# Autodesk Inventor assembly: A2017_T2_05
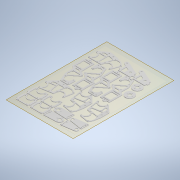
[picture p0: Inventor's stored thumbnail of the model, 180x180]
Saved by Autodesk Inventor 2020 (Build 240168000, 168)
## iProperties
Created: 2021-08-27
Part Number: A2017_T2_05
Document SubType Name: Assembly
Designer: Masato
Author: Masato
## Documents named in this file (9)
- C:\Users\naoki\Documents\Inventor\CitBrains\git_clone\SUSTAINA_ver1_0\AT4_174\SUSTAINA-OP\Cam\A2017_T2_05.iam
- C:\Users\naoki\Documents\Inventor\CitBrains\git_clone\SUSTAINA_ver1_0\AT4_174\SUSTAINA-OP\Cam\DisposableBoard.ipt
- C:\Users\naoki\Documents\Inventor\CitBrains\git_clone\SUSTAINA_ver1_0\AT4_174\SUSTAINA-OP\LowerBody\Ankle\Ankle_back_frame.ipt
- C:\Users\naoki\Documents\Inventor\CitBrains\git_clone\SUSTAINA_ver1_0\AT4_174\SUSTAINA-OP\LowerBody\Foot\Foot_back_frame.ipt
- C:\Users\naoki\Documents\Inventor\CitBrains\git_clone\SUSTAINA_ver1_0\AT4_174\SUSTAINA-OP\LowerBody\Foot\Foot_front_frame.ipt
- C:\Users\naoki\Documents\Inventor\CitBrains\git_clone\SUSTAINA_ver1_0\AT4_174\SUSTAINA-OP\LowerBody\Knee\Knee_side_frame.ipt
- C:\Users\naoki\Documents\Inventor\CitBrains\git_clone\SUSTAINA_ver1_0\AT4_174\SUSTAINA-OP\LowerBody\Leg_joint\Leg_joint_pitch_frame.ipt
- C:\Users\naoki\Documents\Inventor\CitBrains\git_clone\SUSTAINA_ver1_0\AT4_174\SUSTAINA-OP\UpperBody\Trunk\CrossRollerBearing\Inner_flange.ipt
- C:\Users\naoki\Documents\Inventor\CitBrains\git_clone\SUSTAINA_ver1_0\AT4_174\SUSTAINA-OP\LowerBody\Ankle\Ankle_side_frame.ipt
## Components (21 placed, 8 different names)
1. DisposableBoard:1 — メイト:2, メイト:1, フラッシュ:1, フラッシュ:2, メイト:4, フラッシュ:3, フラッシュ:4, メイト:5, メイト:7, メイト:8, メイト:10, 正接:2, メイト:12, メイト:22, メイト:23, メイト:26, メイト:30, メイト:32, メイト:34, メイト:35, メイト:37, メイト:39, 角度:1, メイト:40, 角度:2, 正接:19
2. Foot_back_frame:1 — メイト:5, メイト:9, フラッシュ:5, 正接:1, フラッシュ:6, メイト:28
3. Foot_back_frame:2 — メイト:10, 正接:1, 正接:4, メイト:28
4. Foot_front_frame:1 — メイト:7, フラッシュ:6, 正接:2, 正接:3, メイト:27
5. Foot_front_frame:2 — メイト:8, 正接:3, フラッシュ:8, メイト:27
6. Ankle_side_frame:1 — メイト:22, フラッシュ:13, メイト:25, メイト:29, メイト:41
7. Ankle_side_frame:2 — メイト:23, フラッシュ:12, フラッシュ:13, メイト:25, メイト:33, 正接:12
8. Ankle_side_frame:3 — メイト:26, メイト:29, 正接:9, フラッシュ:14, メイト:31, メイト:36
9. Ankle_side_frame:4 — メイト:30, フラッシュ:14, メイト:31, 正接:15, 正接:16, 正接:17
10. Knee_side_frame:3 — メイト:32, メイト:33, 正接:10, 正接:19
11. Knee_side_frame:4 — メイト:34, 正接:12, メイト:41, 正接:18
12. Leg_joint_pitch_frame:1 — メイト:35, メイト:36, フラッシュ:16, メイト:38, 正接:18
13. Leg_joint_pitch_frame:2 — メイト:37, フラッシュ:16, メイト:38, 正接:14
14. Inner_flange:1 — メイト:39, 正接:14, 正接:15, 角度:1
15. Inner_flange:2 — 正接:16, メイト:40, 角度:2, 正接:17
16. Ankle_back_frame:1 — メイト:4, フラッシュ:3, フラッシュ:4
17. Ankle_back_frame:2 — フラッシュ:12, 正接:10
18. Ankle_back_frame:3 — メイト:9, フラッシュ:5
19. Ankle_back_frame:4
20. Knee_side_frame:1 — メイト:12, フラッシュ:8, 正接:4
21. Knee_side_frame:2 — 正接:9
## Component patterns: (4 elements, first: Ankle_back_frame:1), (2 elements, first: Knee_side_frame:1)
## Relationships (54: Mate 28, Tangent 13, Flush 11, Angle 2)
- メイト:2 [Mate]: DisposableBoard:1
- メイト:1 [Mate]: DisposableBoard:1
- フラッシュ:1 [Flush]: DisposableBoard:1
- フラッシュ:2 [Flush]: DisposableBoard:1
- メイト:4 [Mate]: DisposableBoard:1 ↔ Ankle_back_frame:1
- フラッシュ:3 [Flush] (-2.5 mm): DisposableBoard:1 ↔ Ankle_back_frame:1
- フラッシュ:4 [Flush] (-2.5 mm): DisposableBoard:1 ↔ Ankle_back_frame:1
- メイト:5 [Mate]: DisposableBoard:1 ↔ Foot_back_frame:1
- メイト:7 [Mate]: DisposableBoard:1 ↔ Foot_front_frame:1
- メイト:8 [Mate]: DisposableBoard:1 ↔ Foot_front_frame:2
- メイト:9 [Mate] (2.5 mm): Foot_back_frame:1 ↔ Ankle_back_frame:3
- フラッシュ:5 [Flush]: Foot_back_frame:1 ↔ Ankle_back_frame:3
- メイト:10 [Mate]: DisposableBoard:1 ↔ Foot_back_frame:2
- 正接:1 [Tangent]: Foot_back_frame:1 ↔ Foot_back_frame:2
- フラッシュ:6 [Flush]: Foot_back_frame:1 ↔ Foot_front_frame:1
- 正接:2 [Tangent] (2.5 mm): DisposableBoard:1 ↔ Foot_front_frame:1
- 正接:3 [Tangent]: Foot_front_frame:1 ↔ Foot_front_frame:2
- メイト:12 [Mate]: DisposableBoard:1 ↔ Knee_side_frame:1
- フラッシュ:8 [Flush]: Foot_front_frame:2 ↔ Knee_side_frame:1
- 正接:4 [Tangent] (2.1 mm): Foot_back_frame:2 ↔ Knee_side_frame:1
- メイト:22 [Mate]: DisposableBoard:1 ↔ Ankle_side_frame:1
- メイト:23 [Mate]: DisposableBoard:1 ↔ Ankle_side_frame:2
- フラッシュ:12 [Flush]: Ankle_side_frame:2 ↔ Ankle_back_frame:2
- フラッシュ:13 [Flush]: Ankle_side_frame:1 ↔ Ankle_side_frame:2
- メイト:25 [Mate] (2.5 mm): Ankle_side_frame:1 ↔ Ankle_side_frame:2
- メイト:26 [Mate]: DisposableBoard:1 ↔ Ankle_side_frame:3
- メイト:27 [Mate] (2.5 mm): Foot_front_frame:1 ↔ Foot_front_frame:2
- メイト:28 [Mate] (2.5 mm): Foot_back_frame:1 ↔ Foot_back_frame:2
- メイト:29 [Mate] (2.5 mm): Ankle_side_frame:1 ↔ Ankle_side_frame:3
- 正接:9 [Tangent] (2.5 mm): Ankle_side_frame:3 ↔ Knee_side_frame:2
- メイト:30 [Mate]: DisposableBoard:1 ↔ Ankle_side_frame:4
- フラッシュ:14 [Flush]: Ankle_side_frame:3 ↔ Ankle_side_frame:4
- メイト:31 [Mate] (2.5 mm): Ankle_side_frame:3 ↔ Ankle_side_frame:4
- メイト:32 [Mate]: DisposableBoard:1 ↔ Knee_side_frame:3
- メイト:33 [Mate] (2.5 mm): Ankle_side_frame:2 ↔ Knee_side_frame:3
- 正接:10 [Tangent] (2.5 mm): Knee_side_frame:3 ↔ Ankle_back_frame:2
- メイト:34 [Mate]: DisposableBoard:1 ↔ Knee_side_frame:4
- 正接:12 [Tangent]: Ankle_side_frame:2 ↔ Knee_side_frame:4
- メイト:35 [Mate]: DisposableBoard:1 ↔ Leg_joint_pitch_frame:1
- メイト:36 [Mate] (2.5 mm): Ankle_side_frame:3 ↔ Leg_joint_pitch_frame:1
- メイト:37 [Mate]: DisposableBoard:1 ↔ Leg_joint_pitch_frame:2
- フラッシュ:16 [Flush]: Leg_joint_pitch_frame:1 ↔ Leg_joint_pitch_frame:2
- メイト:38 [Mate] (2.5 mm): Leg_joint_pitch_frame:1 ↔ Leg_joint_pitch_frame:2
- メイト:39 [Mate]: DisposableBoard:1 ↔ Inner_flange:1
- 正接:14 [Tangent] (2.5 mm): Leg_joint_pitch_frame:2 ↔ Inner_flange:1
- 正接:15 [Tangent] (2.5 mm): Ankle_side_frame:4 ↔ Inner_flange:1
- 角度:1 [Angle] (0 deg): DisposableBoard:1 ↔ Inner_flange:1
- 正接:16 [Tangent] (7 mm): Ankle_side_frame:4 ↔ Inner_flange:2
- メイト:40 [Mate]: DisposableBoard:1 ↔ Inner_flange:2
- 角度:2 [Angle] (0 deg): DisposableBoard:1 ↔ Inner_flange:2
- 正接:17 [Tangent] (2.5 mm): Ankle_side_frame:4 ↔ Inner_flange:2
- メイト:41 [Mate] (2.5 mm): Ankle_side_frame:1 ↔ Knee_side_frame:4
- 正接:18 [Tangent] (2.5 mm): Knee_side_frame:4 ↔ Leg_joint_pitch_frame:1
- 正接:19 [Tangent] (2.5 mm): DisposableBoard:1 ↔ Knee_side_frame:3
